# Autodesk Inventor assembly: STM
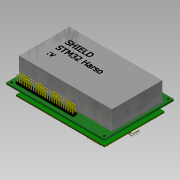
[picture p0: Inventor's stored thumbnail of the model, 180x180]
Saved by Autodesk Inventor 2015 SP1 (Build 190203100, 203)
## iProperties
Created: 2015-02-03
Part Number: STM
Document SubType Name: Assembly
Designer: Rafi Kurnia Putra
Author: Rafi Kurnia Putra
## Documents named in this file (3)
- D:\Dropbox\krpai berkaki trui 2015\ROBUSTA\MEKANIK\ROBUSTA\Assembly STM32 + SHIELD.iam
- D:\Dropbox\krpai berkaki trui 2015\ROBUSTA\MEKANIK\ROBUSTA\SHIELD STM32.ipt
- D:\Dropbox\krpai berkaki trui 2015\ROBUSTA\MEKANIK\ROBUSTA\stm32f4.ipt
## Components (2 placed, 2 different names)
1. SHIELD STM32:1 — Mate:1, Mate:2, Flush:1, Flush:2, Mate:3, Mate:4, Mate:5, Flush:3
2. stm32f4:1 — Mate:1, Mate:2, Flush:1, Flush:2
## Relationships (8: Mate 5, Flush 3)
- Mate:1: SHIELD STM32:1 ↔ stm32f4:1
- Mate:2: SHIELD STM32:1 ↔ stm32f4:1
- Flush:1: SHIELD STM32:1 ↔ stm32f4:1
- Flush:2: SHIELD STM32:1 ↔ stm32f4:1
- Mate:3: SHIELD STM32:1
- Mate:4: SHIELD STM32:1
- Mate:5: SHIELD STM32:1
- Flush:3: SHIELD STM32:1
